# Autodesk Inventor assembly: vehicle assembly v2
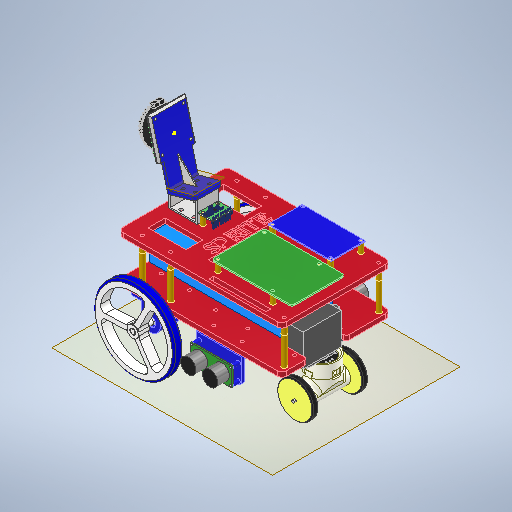
[picture p0: Inventor's stored thumbnail of the model, 512x512]
Saved by Autodesk Inventor 2025.1 (Build 291241020, 241B)
## iProperties
Created: 2024-06-06
Part Number: vehicle assembly v2
Document SubType Name: Assembly
Designer: david
Author: david
## Documents named in this file (30)
- C:\Users\chenc\Downloads\wro_drawings\vehicle assembly v2.iam
- C:\Users\chenc\Downloads\wro_drawings\base plate.ipt
- C:\Users\chenc\Downloads\wro_drawings\bearing holder.ipt
- C:\Users\chenc\Downloads\wro_drawings\servo motor HS-7955TG.iam
- C:\Users\chenc\Downloads\wro_drawings\steering top half.ipt
- steering top half.ipt
- C:\Users\chenc\Downloads\wro_drawings\dfifferential.ipt
- C:\Users\chenc\Downloads\wro_drawings\front wheel.ipt
- C:\Users\chenc\Downloads\wro_drawings\rear wheel 86mm.ipt
- C:\Users\chenc\Downloads\wro_drawings\rear shaft.ipt
- rear shaft.ipt
- C:\Users\chenc\Downloads\wro_drawings\12v DC motor.ipt
- C:\Users\chenc\Downloads\wro_drawings\stand M3-L10.ipt
- C:\Users\chenc\Downloads\wro_drawings\raspberry pi.ipt
- C:\Users\chenc\Downloads\wro_drawings\3s lipo battery.ipt
- C:\Users\chenc\Downloads\wro_drawings\ultrasonic mount.ipt
- C:\Users\chenc\Downloads\wro_drawings\US-015.ipt
- C:\Users\chenc\Downloads\wro_drawings\stand M3-L30.ipt
- C:\Users\chenc\Downloads\wro_drawings\LM2596 Buck Converter.ipt
- C:\Users\chenc\Downloads\wro_drawings\steering bottom half.ipt
- C:\Users\chenc\Downloads\wro_drawings\driver gear adapter v2.ipt
- C:\Users\chenc\Downloads\wro_drawings\ultrasonic mount (front) v2.ipt
- C:\Users\chenc\Downloads\wro_drawings\3S lipo holder v2.ipt
- C:\Users\chenc\Downloads\wro_drawings\12v DC motor mount v2.ipt
- C:\Users\chenc\Downloads\wro_drawings\axle-skibidi-v2.ipt
- C:\Users\chenc\Downloads\wro_drawings\Ramp.ipt
- C:\Users\chenc\Downloads\wro_drawings\top plate modified.ipt
- C:\Users\chenc\Downloads\wro_drawings\Cam + IMU Holder.ipt
- C:\Users\chenc\Downloads\wro_drawings\raspberry-pi-hq-camera\Raspberry Pi HQ Camera\Raspberry Pi HQ Camera\Raspberry Pi HQ Camera.ipt
- C:\Users\chenc\Downloads\wro_drawings\mpu-6050-imu-sensor-1.snapshot.5\MPU 6050 IMU\MPU 6050 IMU\MPU 6050 IMU.ipt
## Components (56 placed, 27 different names)
1. base plate:1 — Insert:60, Insert:61, Insert:62, Insert:63, Mate:9, Mate:10, Mate:11, Flush:6, Flush:7, Flush:8, Insert:74, Insert:75, Insert:134, Insert:135, Insert:136, Insert:137, Insert:138, Insert:139, Insert:140, Insert:141, Insert:196, Insert:197, Insert:198, Insert:199, Insert:200, Insert:201, Insert:202, Insert:203, Mate:19, Insert:208, Insert:209
2. bearing holder:1 — Insert:134, Insert:135, Insert:143
3. bearing holder:2 — Insert:136, Insert:137
4. bearing holder:3 — Insert:140, Insert:141
5. bearing holder:4 — Insert:138, Insert:139, Insert:142
6. dfifferential:1 — Mate:16, Flush:10
7. rear shaft:1 — Insert:83, Angle:9, Insert:143, Mate:16
8. rear shaft:2 — Angle:8, Insert:142, Insert:205
9. rear wheel 86mm:1 — Insert:83, Angle:9
10. rear wheel 86mm:2 — Tangent:1, Angle:8, Insert:205
11. 12v DC motor:1 — Angle:14, Insert:204, Insert:206, Insert:207
12. servo motor HS-7955TG:1 [sub-assembly] — Mate:2, Insert:20, Mate:9, Mate:10, Mate:11
13. steering top half:1 — Insert:20, Mate:14, Mate:15, Angle:12, Angle:13
14. steering bottom half:1 — Mate:14, Mate:15, Angle:12, Insert:210
15. front wheel:1 — Insert:211
16. front wheel:2 — Insert:212
17. stand M3-L30:2 — Insert:60, Insert:150
18. stand M3-L30:3 — Insert:63, Insert:146
19. stand M3-L30:1 — Insert:61, Insert:151
20. stand M3-L30:4 — Insert:62, Insert:148
21. stand M3-L30:9 — Insert:74, Insert:149
22. stand M3-L30:10 — Insert:75, Insert:147
23. stand M3-L10:1 — Insert:169
24. stand M3-L10:2 — Insert:168
25. stand M3-L10:3 — Insert:59
26. stand M3-L10:4 — Insert:58, Insert:219
27. 3s lipo battery:1 — Flush:9, Mate:18, Flush:11
28. ultrasonic mount:1 — Insert:102, Insert:103, Insert:200, Insert:201
29. ultrasonic mount:2 — Insert:106, Insert:107, Insert:198, Insert:199
30. US-015:1 — Insert:102, Insert:103
31. US-015:2 — Insert:106, Insert:107
32. US-015:3 — Insert:194, Insert:195
33. LM2596 Buck Converter:1 — Insert:112, Insert:113, Insert:169, Insert:170
34. stand M3-L10:5 — Insert:167, Insert:220
35. stand M3-L10:6 — Insert:170
36. stand M3-L10:7 — Insert:112, Insert:222
37. stand M3-L10:8 — Insert:113, Insert:221
38. raspberry pi:1 — Insert:58, Insert:59, Insert:167, Insert:168
39. stand M3-L10:9 — Insert:148
40. stand M3-L10:10 — Insert:147
41. stand M3-L10:11 — Insert:151, Insert:217
42. stand M3-L10:12 — Insert:150
43. stand M3-L10:13 — Insert:149
44. stand M3-L10:14 — Insert:146, Insert:218
45. driver gear adapter v2:1 — Angle:14, Insert:204
46. ultrasonic mount (front) v2:1 — Insert:194, Insert:195, Insert:196, Insert:197
47. 3S lipo holder v2:1 — Insert:202, Insert:203, Mate:18, Flush:11
48. 12v DC motor mount v2:1 — Mate:19, Insert:206, Insert:207, Insert:208, Insert:209
49. axle-skibidi-v2:1 — Angle:15, Angle:16, Insert:210, Insert:211, Insert:212
50. Ramp:1 — Insert:215, Insert:216, Insert:223, Insert:224
51. top plate modified:1 — Insert:217, Insert:218, Insert:219, Insert:220, Insert:221, Insert:222, Insert:223, Insert:224, Insert:227, Insert:228
52. Cam + IMU Holder:1 — Insert:215, Insert:216, Insert:225, Insert:226
53. Raspberry Pi HQ Camera:1 — Insert:225, Insert:226
54. MPU 6050 IMU:1 — Insert:229, Insert:230
55. stand M3-L10:15 — Insert:227, Insert:230
56. stand M3-L10:16 — Insert:228, Insert:229
## Relationships (95: Insert 71, Mate 9, Angle 8, Flush 6, Tangent 1)
- Mate:2: servo motor HS-7955TG:1
- Insert:20: servo motor HS-7955TG:1 ↔ steering top half:1
- Angle:4 (0 deg)
- Tangent:1: rear wheel 86mm:2
- Insert:58: stand M3-L10:4 ↔ raspberry pi:1
- Insert:59: stand M3-L10:3 ↔ raspberry pi:1
- Insert:60: base plate:1 ↔ stand M3-L30:2
- Insert:61: base plate:1 ↔ stand M3-L30:1
- Insert:62: base plate:1 ↔ stand M3-L30:4
- Insert:63: base plate:1 ↔ stand M3-L30:3
- Mate:9: base plate:1 ↔ servo motor HS-7955TG:1
- Mate:10: base plate:1 ↔ servo motor HS-7955TG:1
- Mate:11: base plate:1 ↔ servo motor HS-7955TG:1
- Flush:6: base plate:1
- Flush:7: base plate:1
- Flush:8: base plate:1
- Insert:74: base plate:1 ↔ stand M3-L30:9
- Insert:75: base plate:1 ↔ stand M3-L30:10
- Insert:83: rear shaft:1 ↔ rear wheel 86mm:1
- Angle:8 (180 deg): rear shaft:2 ↔ rear wheel 86mm:2
- Angle:9 (180 deg): rear shaft:1 ↔ rear wheel 86mm:1
- Insert:102: ultrasonic mount:1 ↔ US-015:1
- Insert:103: ultrasonic mount:1 ↔ US-015:1
- Insert:106: ultrasonic mount:2 ↔ US-015:2
- Insert:107: ultrasonic mount:2 ↔ US-015:2
- Insert:112: LM2596 Buck Converter:1 ↔ stand M3-L10:7
- Insert:113: LM2596 Buck Converter:1 ↔ stand M3-L10:8
- Insert:134: base plate:1 ↔ bearing holder:1
- Insert:135: base plate:1 ↔ bearing holder:1
- Insert:136: base plate:1 ↔ bearing holder:2
- Insert:137: base plate:1 ↔ bearing holder:2
- Insert:138: base plate:1 ↔ bearing holder:4
- Insert:139: base plate:1 ↔ bearing holder:4
- Insert:140: base plate:1 ↔ bearing holder:3
- Insert:141: base plate:1 ↔ bearing holder:3
- Insert:142: bearing holder:4 ↔ rear shaft:2
- Insert:143: bearing holder:1 ↔ rear shaft:1
- Insert:146: stand M3-L30:3 ↔ stand M3-L10:14
- Insert:147: stand M3-L30:10 ↔ stand M3-L10:10
- Insert:148: stand M3-L30:4 ↔ stand M3-L10:9
- Insert:149: stand M3-L30:9 ↔ stand M3-L10:13
- Insert:150: stand M3-L30:2 ↔ stand M3-L10:12
- Insert:151: stand M3-L30:1 ↔ stand M3-L10:11
- Flush:9: 3s lipo battery:1
- Mate:14: steering top half:1 ↔ steering bottom half:1
- Mate:15: steering top half:1 ↔ steering bottom half:1
- Angle:12 (180 deg): steering top half:1 ↔ steering bottom half:1
- Angle:13 (0 deg): steering top half:1
- Insert:167: stand M3-L10:5 ↔ raspberry pi:1
- Insert:168: stand M3-L10:2 ↔ raspberry pi:1
- Insert:169: stand M3-L10:1 ↔ LM2596 Buck Converter:1
- Insert:170: LM2596 Buck Converter:1 ↔ stand M3-L10:6
- Mate:16: dfifferential:1 ↔ rear shaft:1
- Flush:10: dfifferential:1
- Insert:194: US-015:3 ↔ ultrasonic mount (front) v2:1
- Insert:195: US-015:3 ↔ ultrasonic mount (front) v2:1
- Insert:196: base plate:1 ↔ ultrasonic mount (front) v2:1
- Insert:197: base plate:1 ↔ ultrasonic mount (front) v2:1
- Insert:198: base plate:1 ↔ ultrasonic mount:2
- Insert:199: base plate:1 ↔ ultrasonic mount:2
- Insert:200: base plate:1 ↔ ultrasonic mount:1
- Insert:201: base plate:1 ↔ ultrasonic mount:1
- Insert:202: base plate:1 ↔ 3S lipo holder v2:1
- Insert:203: base plate:1 ↔ 3S lipo holder v2:1
- Mate:18 (-3 mm): 3s lipo battery:1 ↔ 3S lipo holder v2:1
- Angle:14 (180 deg): 12v DC motor:1 ↔ driver gear adapter v2:1
- Insert:204: 12v DC motor:1 ↔ driver gear adapter v2:1
- Flush:11: 3s lipo battery:1 ↔ 3S lipo holder v2:1
- Insert:205: rear shaft:2 ↔ rear wheel 86mm:2
- Mate:19: base plate:1 ↔ 12v DC motor mount v2:1
- Insert:206: 12v DC motor:1 ↔ 12v DC motor mount v2:1
- Insert:207: 12v DC motor:1 ↔ 12v DC motor mount v2:1
- Insert:208: base plate:1 ↔ 12v DC motor mount v2:1
- Insert:209: base plate:1 ↔ 12v DC motor mount v2:1
- Angle:15 (0 deg): axle-skibidi-v2:1
- Angle:16 (180 deg): axle-skibidi-v2:1
- Insert:210: steering bottom half:1 ↔ axle-skibidi-v2:1
- Insert:211 (2 mm): front wheel:1 ↔ axle-skibidi-v2:1
- Insert:212 (2 mm): front wheel:2 ↔ axle-skibidi-v2:1
- Insert:215: Ramp:1 ↔ Cam + IMU Holder:1
- Insert:216: Ramp:1 ↔ Cam + IMU Holder:1
- Insert:217: stand M3-L10:11 ↔ top plate modified:1
- Insert:218: stand M3-L10:14 ↔ top plate modified:1
- Insert:219: stand M3-L10:4 ↔ top plate modified:1
- Insert:220: stand M3-L10:5 ↔ top plate modified:1
- Insert:221: stand M3-L10:8 ↔ top plate modified:1
- Insert:222: stand M3-L10:7 ↔ top plate modified:1
- Insert:223: Ramp:1 ↔ top plate modified:1
- Insert:224: Ramp:1 ↔ top plate modified:1
- Insert:225: Cam + IMU Holder:1 ↔ Raspberry Pi HQ Camera:1
- Insert:226: Cam + IMU Holder:1 ↔ Raspberry Pi HQ Camera:1
- Insert:227: top plate modified:1 ↔ stand M3-L10:15
- Insert:228: top plate modified:1 ↔ stand M3-L10:16
- Insert:229: MPU 6050 IMU:1 ↔ stand M3-L10:16
- Insert:230: MPU 6050 IMU:1 ↔ stand M3-L10:15
